# Autodesk Inventor assembly: Packing Nut Subassembly
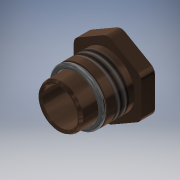
[picture p0: Inventor's stored thumbnail of the model, 180x180]
Saved by Autodesk Inventor 2018 (Build 220112000, 112)
## iProperties
Created: 2017-10-19
Part Number: Packing Nut Subassembly
Document SubType Name: Assembly
Designer: kurtis
Author: kurtis
## Documents named in this file (4)
- D:\Users\kurti\Git-Home\CAD\GE101\MA6\Packing Nut Subassembly.iam
- D:\Users\kurti\Git-Home\CAD\GE101\MA6\Oring3.ipt
- D:\Users\kurti\Git-Home\CAD\GE101\MA6\Packing Nut.ipt
- D:\Users\kurti\Git-Home\CAD\GE101\MA6\Oring2.ipt
## Components (3 placed, 3 different names)
1. Oring3:1 — Rigid:1
2. Packing Nut:1 — Rigid:1, Rigid:2
3. Oring2:1 — Rigid:2
## Relationships (2: WeldJoint 2)
- Rigid:1 [WeldJoint] (1 mm): Oring3:1 ↔ Packing Nut:1
- Rigid:2 [WeldJoint] (1 mm): Packing Nut:1 ↔ Oring2:1
